# Autodesk Inventor assembly: HS 60T Gear, Circle Insert
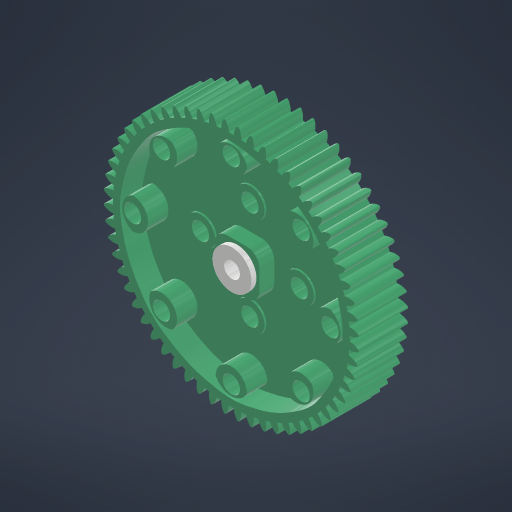
[picture p0: Inventor's stored thumbnail of the model, 512x512]
Saved by Autodesk Inventor 2024 (Build 280153000, 153)
## iProperties
Created: 2023-08-12
Part Number: HS 60T Gear, Circle Insert
Document SubType Name: Assembly
Designer: macbook
Author: macbook
## Documents named in this file (3)
- \\Mac\Home\Desktop\code\7899V-VRC-OVER-UNDER\Cad\VEX-CAD-Inventor-1.4.0\Motion\Gears\HS Gear\HS 60T Gear, Circle Insert.iam
- \\Mac\Home\Desktop\code\7899V-VRC-OVER-UNDER\Cad\VEX-CAD-Inventor-1.4.0\Motion\Insert Circle.ipt
- \\Mac\Home\Desktop\code\7899V-VRC-OVER-UNDER\Cad\VEX-CAD-Inventor-1.4.0\Motion\Gears\60T_High_Strength_Gear_276-5035\60T_High_Strength_Gear_276-5035.ipt
## Components (3 placed, 2 different names)
1. Insert Circle:1 — Mate:3, Mate:4, Mate:5
2. Insert Circle:2 — Mate:1, Mate:2, Mate:6
3. 60T_High_Strength_Gear_276-5035:1 — Mate:1, Mate:2, Mate:3, Mate:4, Mate:5, Mate:6
## Relationships (6: Mate 6)
- Mate:1: Insert Circle:2 ↔ 60T_High_Strength_Gear_276-5035:1
- Mate:2: Insert Circle:2 ↔ 60T_High_Strength_Gear_276-5035:1
- Mate:3: Insert Circle:1 ↔ 60T_High_Strength_Gear_276-5035:1
- Mate:4: Insert Circle:1 ↔ 60T_High_Strength_Gear_276-5035:1
- Mate:5: Insert Circle:1 ↔ 60T_High_Strength_Gear_276-5035:1
- Mate:6: Insert Circle:2 ↔ 60T_High_Strength_Gear_276-5035:1
